# Autodesk Inventor assembly: Assembly1
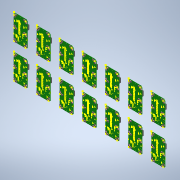
[picture p0: Inventor's stored thumbnail of the model, 180x180]
Saved by Autodesk Inventor 2020 (Build 240168000, 168)
## iProperties
Created: 2020-07-08
Part Number: Assembly1
Document SubType Name: Assembly
Designer: gerac
Author: gerac
## Documents named in this file (2)
- C:\Users\gerac\Desktop\HES-SO_3\BACHELOR_THESIS\HypnosiaControllerGIT\HYPNOSIA_Inventor\Assembly1.iam
- C:\Users\gerac\Desktop\HES-SO_3\BACHELOR_THESIS\HypnosiaControllerGIT\HYPNOSIA_Inventor\HYPNOSIA_V2.iam
## Components (14 placed, 1 different names)
1. HYPNOSIA_V2:1 [sub-assembly]
2. HYPNOSIA_V2:2 [sub-assembly]
3. HYPNOSIA_V2:3 [sub-assembly]
4. HYPNOSIA_V2:4 [sub-assembly]
5. HYPNOSIA_V2:5 [sub-assembly]
6. HYPNOSIA_V2:6 [sub-assembly]
7. HYPNOSIA_V2:7 [sub-assembly]
8. HYPNOSIA_V2:8 [sub-assembly]
9. HYPNOSIA_V2:9 [sub-assembly]
10. HYPNOSIA_V2:10 [sub-assembly]
11. HYPNOSIA_V2:11 [sub-assembly]
12. HYPNOSIA_V2:12 [sub-assembly]
13. HYPNOSIA_V2:13 [sub-assembly]
14. HYPNOSIA_V2:14 [sub-assembly]
## Component patterns: (14 elements, first: HYPNOSIA_V2:1)
